# Autodesk Inventor assembly: Gear_test_1
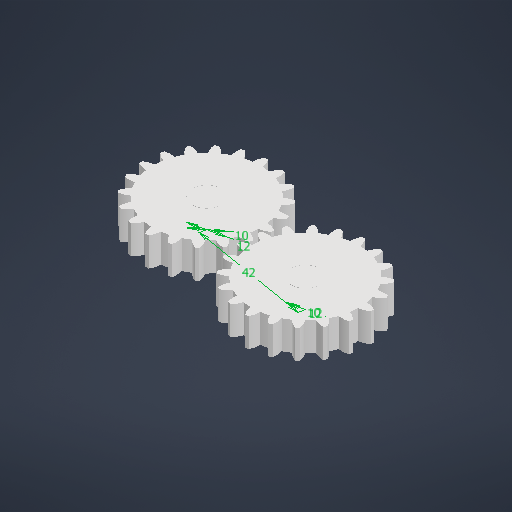
[picture p0: Inventor's stored thumbnail of the model, 512x512]
Saved by Autodesk Inventor 2026.2 (Build 302298000, 298)
## iProperties
Created: 2025-12-17
Part Number: Gear_test_1
Document SubType Name: Assembly
Designer: Cobble
Author: Cobble
## Documents named in this file (3)
- D:\CAD\Gear_test_1.iam
- D:\CAD\Test.ipt
- D:\CAD\40mm_20N_Gear.ipt
## Components (3 placed, 2 different names)
1. Test:1 — Insert:1, Insert:2
2. 40mm_20N_Gear:1 — Insert:1, Rotation:1
3. 40mm_20N_Gear:2 — Insert:2, Rotation:1
## Relationships (3: Insert 2, RelateRotation 1)
- Insert:1: Test:1 ↔ 40mm_20N_Gear:1
- Insert:2: Test:1 ↔ 40mm_20N_Gear:2
- Rotation:1 [RelateRotation] (-1 ul): 40mm_20N_Gear:1 ↔ 40mm_20N_Gear:2
